# Autodesk Inventor assembly: Assembly1
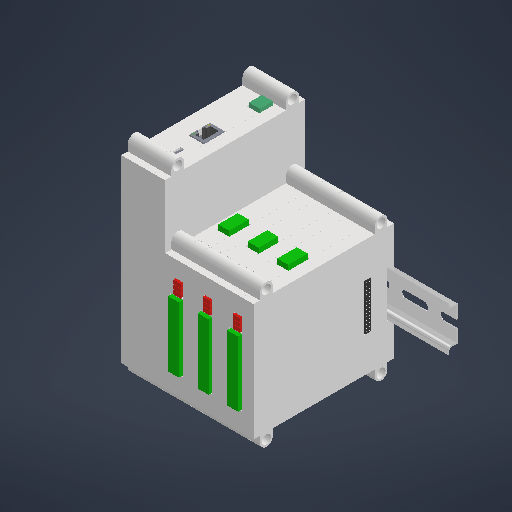
[picture p0: Inventor's stored thumbnail of the model, 512x512]
Saved by Autodesk Inventor 2025 (Build 290162000, 162)
## iProperties
Created: 2024-08-31
Part Number: Assembly1
Document SubType Name: Assembly
Designer: Dawid
Author: Dawid
## Documents named in this file (4)
- C:\Users\Dawid\Desktop\Magisterka\plc_io_module_case\Assembly1.iam
- C:\Users\Dawid\Desktop\Magisterka\plc_io_module_case\din_rail.ipt
- C:\Users\Dawid\Desktop\Magisterka\plc_io_module_case\module.iam
- C:\Users\Dawid\Desktop\Magisterka\plc_io_module_case\cpu_module.iam
## Components (5 placed, 3 different names)
1. din_rail.ipt:1 — Slider:1, Slider:2, Slider:3, Slider:4
2. module.iam:1 [sub-assembly] — Slider:1, Mate:1, Mate:2
3. module.iam:2 [sub-assembly] — Slider:3, Mate:2, Mate:3
4. module.iam:3 [sub-assembly] — Slider:2, Mate:3
5. cpu_module:1 [sub-assembly] — Slider:4, Mate:1
## Relationships (7: TranslationJoint 4, Mate 3)
- Slider:1 [TranslationJoint]: din_rail.ipt:1 ↔ module.iam:1
- Slider:2 [TranslationJoint]: din_rail.ipt:1 ↔ module.iam:3
- Slider:3 [TranslationJoint]: din_rail.ipt:1 ↔ module.iam:2
- Slider:4 [TranslationJoint]: din_rail.ipt:1 ↔ cpu_module:1
- Mate:1: module.iam:1 ↔ cpu_module:1
- Mate:2: module.iam:1 ↔ module.iam:2
- Mate:3: module.iam:2 ↔ module.iam:3
